# Autodesk Inventor assembly: Trs_Aereo
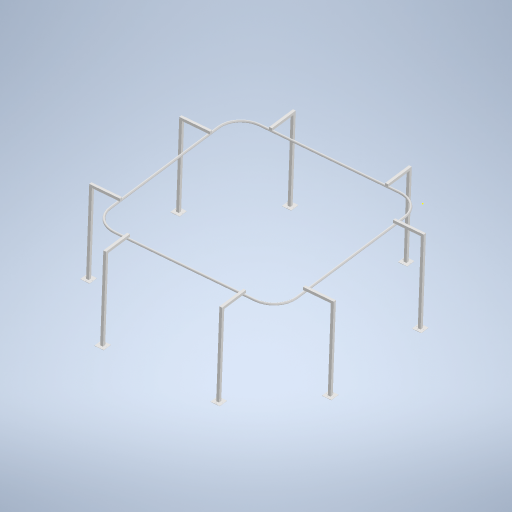
[picture p0: Inventor's stored thumbnail of the model, 512x512]
Saved by Autodesk Inventor 2024 (Build 280153000, 153)
## iProperties
Created: 2023-04-22
Part Number: Trs_Aereo
Document SubType Name: Assembly
Designer: javie
Author: javie
## Documents named in this file (3)
- C:\Users\javie\Downloads\Trs_Aereo.iam
- C:\Users\javie\Downloads\Sriel.ipt
- C:\Users\javie\Downloads\Riel.ipt
## Components (9 placed, 2 different names)
1. Sriel:1 — Rígido:1
2. Riel:1 — Rígido:1, Rígido:4, Rígido:2, Rígido:3, Rígido:8, Rígido:5, Rígido:6, Rígido:7
3. Sriel:2 — Rígido:4
4. Sriel:3 — Rígido:2
5. Sriel:4 — Rígido:3
6. Sriel:5 — Rígido:8
7. Sriel:6 — Rígido:5
8. Sriel:7 — Rígido:7
9. Sriel:8 — Rígido:6
## Relationships (8: WeldJoint 8)
- Rígido:1 [WeldJoint] (-254 mm): Sriel:1 ↔ Riel:1
- Rígido:4 [WeldJoint] (254 mm): Riel:1 ↔ Sriel:2
- Rígido:2 [WeldJoint] (-254 mm): Riel:1 ↔ Sriel:3
- Rígido:3 [WeldJoint] (254 mm): Riel:1 ↔ Sriel:4
- Rígido:8 [WeldJoint] (-254 mm): Riel:1 ↔ Sriel:5
- Rígido:5 [WeldJoint] (254 mm): Riel:1 ↔ Sriel:6
- Rígido:6 [WeldJoint] (-254 mm): Riel:1 ↔ Sriel:8
- Rígido:7 [WeldJoint] (254 mm): Riel:1 ↔ Sriel:7
